# Autodesk Inventor assembly: Clamex Joint
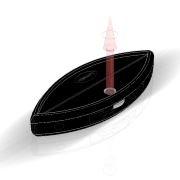
[picture p0: Inventor's stored thumbnail of the model, 180x180]
Saved by Autodesk Inventor 2022.5 (Build 265521000, 521)
## iProperties
RuleStatus: InUse
Created: 2023-01-31
Part Number: Clamex Joint
Document SubType Name: Assembly
Designer: sauliusd
Author: sauliusd
## Documents named in this file (3)
- D:\W4INV 2022 Design\SMART HARDWARE\Lamello Clamex P-10 Joint\Lamello Clamex P10 Joint.iam
- D:\W4INV 2022 Design\SMART HARDWARE\Lamello Clamex P-10 Joint\Parts\Clamex Joint P-10.ipt
- D:\W4INV 2022 Design\LIBRARY\Fixed joints\Lamello Clamex P-10\Clamex P-10 Connector.iam
## Components (3 placed, 3 different names)
1. @Skeleton — Mate:1, Flush:1, Flush:3
2. Clamex P-14 Lammelo — Mate:1, Flush:1
3. Clamex P-10 Connector:2 [sub-assembly]
## Component patterns: (2 elements, first: Clamex P-14 Lammelo)
## Relationships (3: Flush 2, Mate 1)
- Mate:1: @Skeleton ↔ Clamex P-14 Lammelo
- Flush:1: @Skeleton ↔ Clamex P-14 Lammelo
- Flush:3: @Skeleton
## Named parameters: ContactPatchWidth = 300 mm, ContactPatchHeight = 18 mm, ConnectionAngle = 80 deg, NestledBoardT = 18 mm, PillarBoardT = 18 mm, MinDistFromSide = 50 mm, SideDist1 = 60 mm, MaxDistBetween = 480 mm, SideDist2 = 60 mm, MaxDistFromSide = 180 mm, ShiftY = 0 mm, Gap = 0 mm
